# Autodesk Inventor assembly: Dichtung
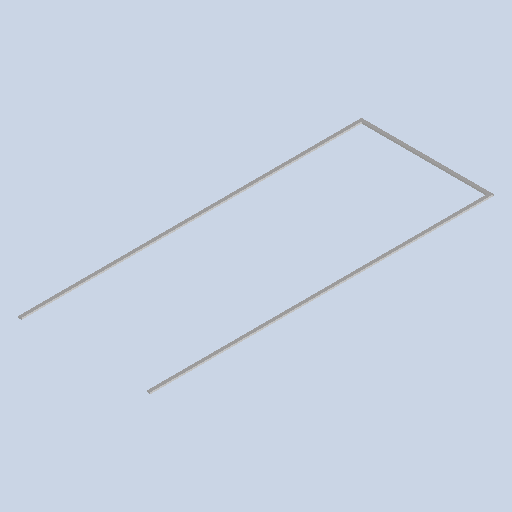
[picture p0: Inventor's stored thumbnail of the model, 512x512]
Saved by Autodesk Inventor 2025.1 (Build 291241000, 241)
## iProperties
Created: 2024-08-07
Part Number: Dichtung
Document SubType Name: Assembly
Designer: ffogue
Author: ffogue
## Documents named in this file (4)
- C:\Users\ffogue\Documents\Inventor\BrandschutzTuer\Dichtung.iam
- C:\Users\ffogue\Documents\Inventor\BrandschutzTuer\Dichtung_links.ipt
- C:\Users\ffogue\Documents\Inventor\BrandschutzTuer\DitchtungRahmen.ipt
- C:\Users\ffogue\Documents\Inventor\BrandschutzTuer\Dichtung_Rechts.ipt
## Components (3 placed, 3 different names)
1. Dichtung_links:1 — Flush:1, Mate:1
2. DitchtungRahmen:1 — Flush:1, Mate:1, Flush:2, Mate:2
3. Dichtung_Rechts:1 — Flush:2, Mate:2
## Relationships (4: Flush 2, Mate 2)
- Flush:1: Dichtung_links:1 ↔ DitchtungRahmen:1
- Mate:1: Dichtung_links:1 ↔ DitchtungRahmen:1
- Flush:2: DitchtungRahmen:1 ↔ Dichtung_Rechts:1
- Mate:2: DitchtungRahmen:1 ↔ Dichtung_Rechts:1
